# Autodesk Inventor assembly: Framework_Link_COG
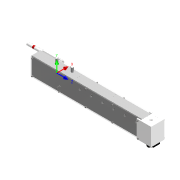
[picture p0: Inventor's stored thumbnail of the model, 180x180]
Saved by Autodesk Inventor 2022 (Build 260153000, 153)
## iProperties
Created: 2022-10-18
Part Number: Framework_Link_COG
Document SubType Name: Assembly
Designer: alexw
Mass: 1238.25 g
Surface Area: 4599.21 cm^2
Volume: 1168.94 cm^3
Density: 1.05929 g/cm^3
Author: alexw
## Documents named in this file (17)
- C:\Users\alexw\Documents\Inventor\Projects\03_CurrentProjects\MasterThesis\PSM_V1_Rillenkugellager\COG\Framework_Link_COG.iam
- C:\Users\alexw\Documents\Inventor\Projects\03_CurrentProjects\MasterThesis\PSM_V1_Rillenkugellager\Ueberarbeiteter DaVincikopf\Fuehrungsschiene.ipt
- C:\Users\alexw\Documents\Inventor\Projects\03_CurrentProjects\MasterThesis\PSM_V1_Rillenkugellager\Back plate profile.ipt
- C:\Users\alexw\Documents\Inventor\Projects\03_CurrentProjects\MasterThesis\PSM_V1_Rillenkugellager\Slot profile.ipt
- C:\Users\alexw\Documents\Inventor\Projects\03_CurrentProjects\MasterThesis\PSM_V1_Rillenkugellager\Guide.ipt
- C:\Users\alexw\Documents\Inventor\Projects\03_CurrentProjects\MasterThesis\PSM_V1_Rillenkugellager\Ueberarbeiteter DaVincikopf\Zahnradbahn.ipt
- C:\Users\alexw\Documents\Inventor\Projects\03_CurrentProjects\MasterThesis\PSM_V1_Rillenkugellager\ContentCenter\de-DE\ISO 4762(2)\ISO 4762 - M3 x 10ISO.ipt
- C:\Users\alexw\Documents\Inventor\Projects\03_CurrentProjects\MasterThesis\PSM_V1_Rillenkugellager\ContentCenter\de-DE\ISO 4762(2)\ISO 4762 - M3 x 12ISO.ipt
- C:\Users\alexw\Documents\Inventor\Projects\03_CurrentProjects\MasterThesis\PSM_V1_Rillenkugellager\ContentCenter\de-DE\ISO 10642(1)\ISO 10642 - M3 x  8.ipt
- C:\Users\alexw\Documents\Inventor\Projects\03_CurrentProjects\MasterThesis\PSM_V1_Rillenkugellager\ContentCenter\de-DE\ISO 4762(2)\ISO 4762 - M3 x 16ISO.ipt
- C:\Users\alexw\Documents\Inventor\Projects\03_CurrentProjects\MasterThesis\PSM_V1_Rillenkugellager\Riemenspanner_Bottompart_Assembly.iam
- C:\Users\alexw\Documents\Inventor\Projects\03_CurrentProjects\MasterThesis\PSM_V1_Rillenkugellager\Sensor_Box_Assembly.ipt.iam
- C:\Users\alexw\Documents\Inventor\Projects\03_CurrentProjects\MasterThesis\PSM_V1_Rillenkugellager\ContentCenter\de-DE\ISO 4762(2)\ISO 4762 - M3 x 20ISO.ipt
- C:\Users\alexw\Documents\Inventor\Projects\03_CurrentProjects\MasterThesis\PSM_V1_Rillenkugellager\Riemen_T5.ipt
- C:\Users\alexw\Documents\Inventor\Projects\03_CurrentProjects\MasterThesis\PSM_V1_Rillenkugellager\ContentCenter\de-DE\ISO 4762(2)\ISO 4762 - M5 x 25ISO.ipt
- C:\Users\alexw\Documents\Inventor\Projects\03_CurrentProjects\MasterThesis\PSM_V1_Rillenkugellager\10_79_0000_0010_003.ipt
- Sensor_Box_Assembly.ipt
## Components (43 placed, 15 different names)
1. Fuehrungsschiene:1 — Passend:73, Passend:74, Passend:75, Passend:76, Passend:77, Passend:78, Passend:79, Passend:80, Fluchtend:3
2. Back plate profile:1 — Winkel:1
3. Slot profile:1
4. Guide:1
5. Zahnradbahn:1
6. ISO 4762 M3 x 10:1
7. ISO 4762 M3 x 10:2
8. ISO 4762 M3 x 10:3
9. ISO 4762 M3 x 10:4
10. ISO 4762 M3 x 10:5
11. ISO 4762 M3 x 10:6
12. ISO 4762 M3 x 10:7
13. ISO 4762 M3 x 10:8
14. ISO 4762 M3 x 12:1
15. ISO 4762 M3 x 12:2
16. ISO 4762 M3 x 12:3
17. ISO 4762 M3 x 12:4
18. ISO 4762 M3 x 12:5
19. ISO 4762 M3 x 12:6
20. ISO 10642 M3x8:1
21. ISO 10642 M3x8:2
22. ISO 10642 M3x8:3
23. ISO 10642 M3x8:4
24. ISO 10642 M3x8:5
25. ISO 10642 M3x8:6
26. ISO 4762 M3 x 16:1
27. ISO 4762 M3 x 16:2
28. ISO 4762 M3 x 16:3
29. ISO 4762 M3 x 16:4
30. Riemenspanner_Bottompart_Assembly:1 [sub-assembly] — Passend:83
31. Sensor_Box_Assembly.ipt:1 [sub-assembly] — Passend:84
32. ISO 4762 M3 x 20:1
33. ISO 4762 M3 x 20:2
34. ISO 4762 M3 x 20:3
35. ISO 4762 M3 x 20:4
36. ISO 4762 M3 x 16:5
37. ISO 4762 M3 x 16:6
38. Riemen_T5:1 — Passend:83, Passend:84
39. ISO 4762 M5 x 25:1
40. 10_79_0000_0010_003:1 — Passend:73, Passend:79
41. 10_79_0000_0010_003:2 — Passend:74, Passend:80, Passend:81, Passend:82
42. 10_79_0000_0010_003:3 — Passend:75, Passend:77
43. 10_79_0000_0010_003:4 — Passend:76, Passend:78
## Relationships (88: Mate 84, Flush 3, Angle 1)
- [Mate]: Fuehrungsschiene:1 ↔ Slot profile:1
- [Mate]: Slot profile:1 ↔ Guide:1
- [Mate]: Fuehrungsschiene:1 ↔ ISO 4762 M3 x 10:1
- [Mate]: Back plate profile:1 ↔ ISO 4762 M3 x 10:1
- [Mate]: Fuehrungsschiene:1 ↔ ISO 4762 M3 x 10:2
- [Mate]: Back plate profile:1 ↔ ISO 4762 M3 x 10:2
- [Mate]: Fuehrungsschiene:1 ↔ ISO 4762 M3 x 10:3
- [Mate]: Back plate profile:1 ↔ ISO 4762 M3 x 10:3
- [Mate]: Fuehrungsschiene:1 ↔ ISO 4762 M3 x 10:4
- [Mate]: Back plate profile:1 ↔ ISO 4762 M3 x 10:4
- [Mate]: Fuehrungsschiene:1 ↔ ISO 4762 M3 x 10:5
- [Mate]: Back plate profile:1 ↔ ISO 4762 M3 x 10:5
- [Mate]: Fuehrungsschiene:1 ↔ ISO 4762 M3 x 10:6
- [Mate]: Back plate profile:1 ↔ ISO 4762 M3 x 10:6
- [Mate]: Fuehrungsschiene:1 ↔ ISO 4762 M3 x 10:7
- [Mate]: Back plate profile:1 ↔ ISO 4762 M3 x 10:7
- [Mate]: Fuehrungsschiene:1 ↔ ISO 4762 M3 x 10:8
- [Mate]: Back plate profile:1 ↔ ISO 4762 M3 x 10:8
- [Mate]: Fuehrungsschiene:1 ↔ ISO 4762 M3 x 12:1
- [Mate]: Slot profile:1 ↔ ISO 4762 M3 x 12:1
- [Mate]: Fuehrungsschiene:1 ↔ ISO 4762 M3 x 12:2
- [Mate]: Slot profile:1 ↔ ISO 4762 M3 x 12:2
- [Mate]: Fuehrungsschiene:1 ↔ ISO 4762 M3 x 12:3
- [Mate]: Slot profile:1 ↔ ISO 4762 M3 x 12:3
- [Mate]: Fuehrungsschiene:1 ↔ ISO 4762 M3 x 12:4
- [Mate]: Slot profile:1 ↔ ISO 4762 M3 x 12:4
- [Mate]: Fuehrungsschiene:1 ↔ ISO 4762 M3 x 12:5
- [Mate]: Slot profile:1 ↔ ISO 4762 M3 x 12:5
- [Mate]: Fuehrungsschiene:1 ↔ ISO 4762 M3 x 12:6
- [Mate]: Slot profile:1 ↔ ISO 4762 M3 x 12:6
- [Mate]: Fuehrungsschiene:1 ↔ Back plate profile:1
- [Mate]: Back plate profile:1 ↔ ISO 4762 M3 x 10:7
- [Mate]: Fuehrungsschiene:1 ↔ Slot profile:1
- [Mate]: Fuehrungsschiene:1 ↔ ISO 10642 M3x8:1
- [Mate]: Fuehrungsschiene:1 ↔ ISO 10642 M3x8:2
- [Mate]: Fuehrungsschiene:1 ↔ ISO 10642 M3x8:3
- [Mate]: Fuehrungsschiene:1 ↔ ISO 10642 M3x8:4
- [Mate]: Fuehrungsschiene:1 ↔ ISO 10642 M3x8:5
- [Mate]: Fuehrungsschiene:1 ↔ ISO 10642 M3x8:6
- [Mate]: Slot profile:1 ↔ Guide:1
- [Mate]: Slot profile:1 ↔ Guide:1
- [Mate]: Fuehrungsschiene:1 ↔ Zahnradbahn:1
- [Flush]: Fuehrungsschiene:1 ↔ Zahnradbahn:1
- [Mate]: Fuehrungsschiene:1 ↔ Zahnradbahn:1
- [Mate]: Fuehrungsschiene:1 ↔ Zahnradbahn:1
- [Mate]: Guide:1 ↔ ISO 4762 M3 x 16:1
- [Mate]: Guide:1 ↔ ISO 4762 M3 x 16:1
- [Mate]: Guide:1 ↔ ISO 4762 M3 x 16:2
- [Mate]: Guide:1 ↔ ISO 4762 M3 x 16:2
- [Mate]: Guide:1 ↔ ISO 4762 M3 x 16:3
- [Mate]: Guide:1 ↔ ISO 4762 M3 x 16:3
- [Mate]: Guide:1 ↔ ISO 4762 M3 x 16:4
- [Mate]: Guide:1 ↔ ISO 4762 M3 x 16:4
- [Mate]: Fuehrungsschiene:1 ↔ Riemenspanner_Bottompart_Assembly:1
- [Mate]: Fuehrungsschiene:1 ↔ Riemenspanner_Bottompart_Assembly:1
- [Mate]: Back plate profile:1 ↔ Sensor_Box_Assembly.ipt:1
- [Mate]: Fuehrungsschiene:1 ↔ Sensor_Box_Assembly.ipt:1
- [Mate]: Slot profile:1 ↔ Sensor_Box_Assembly.ipt:1
- [Mate]: Fuehrungsschiene:1 ↔ ISO 4762 M3 x 20:1
- [Mate]: Sensor_Box_Assembly.ipt:1 ↔ ISO 4762 M3 x 20:1
- [Mate]: Sensor_Box_Assembly.ipt:1 ↔ ISO 4762 M3 x 20:2
- [Mate]: Sensor_Box_Assembly.ipt:1 ↔ ISO 4762 M3 x 20:2
- [Mate]: Sensor_Box_Assembly.ipt:1 ↔ ISO 4762 M3 x 20:3
- [Mate]: Sensor_Box_Assembly.ipt:1 ↔ ISO 4762 M3 x 20:3
- [Mate]: Sensor_Box_Assembly.ipt:1 ↔ ISO 4762 M3 x 20:4
- [Mate]: Sensor_Box_Assembly.ipt:1 ↔ ISO 4762 M3 x 20:4
- [Mate]: Sensor_Box_Assembly.ipt:1 ↔ ISO 4762 M3 x 16:5
- [Mate]: Sensor_Box_Assembly.ipt:1 ↔ ISO 4762 M3 x 16:5
- [Mate]: Sensor_Box_Assembly.ipt:1 ↔ ISO 4762 M3 x 16:6
- [Mate]: Sensor_Box_Assembly.ipt:1 ↔ ISO 4762 M3 x 16:6
- [Mate] (370 mm): Riemenspanner_Bottompart_Assembly:1 ↔ Sensor_Box_Assembly.ipt:1
- [Mate]: Fuehrungsschiene:1 ↔ ISO 4762 M5 x 25:1
- [Mate]: Riemenspanner_Bottompart_Assembly:1 ↔ ISO 4762 M5 x 25:1
- [Flush]: Sensor_Box_Assembly.ipt:1 ↔ Riemen_T5:1
- Passend:73 [Mate]: Fuehrungsschiene:1 ↔ 10_79_0000_0010_003:1
- Passend:74 [Mate]: Fuehrungsschiene:1 ↔ 10_79_0000_0010_003:2
- Passend:75 [Mate]: Fuehrungsschiene:1 ↔ 10_79_0000_0010_003:3
- Passend:76 [Mate]: Fuehrungsschiene:1 ↔ 10_79_0000_0010_003:4
- Passend:77 [Mate]: Fuehrungsschiene:1 ↔ 10_79_0000_0010_003:3
- Passend:78 [Mate]: Fuehrungsschiene:1 ↔ 10_79_0000_0010_003:4
- Passend:79 [Mate]: Fuehrungsschiene:1 ↔ 10_79_0000_0010_003:1
- Passend:80 [Mate]: Fuehrungsschiene:1 ↔ 10_79_0000_0010_003:2
- Passend:81 [Mate]: 10_79_0000_0010_003:2
- Passend:82 [Mate]: 10_79_0000_0010_003:2
- Winkel:1 [Angle] (0 deg): Back plate profile:1
- Passend:83 [Mate]: Riemenspanner_Bottompart_Assembly:1 ↔ Riemen_T5:1
- Passend:84 [Mate]: Sensor_Box_Assembly.ipt:1 ↔ Riemen_T5:1
- Fluchtend:3 [Flush]: Fuehrungsschiene:1
## Named parameters: d85_d117 = 0 mm, d86_d118 = 0 mm, d87_d119 = 0 mm, d88_d120 = 0 mm, d89_d121 = 0 mm, d90_d122 = 0 mm, d91_d123 = 0 mm, d92_d124 = 0 mm, d93_d125 = 0 mm, d94_d126 = 0 mm, d95_d127 = 0 mm, d96_d128 = 0 mm, d97_d129 = 0 mm, d98_d130 = 0 mm, d99_d131 = 0 mm, d100_d132 = 0 mm, d101_d133 = 0 mm, d102_d134 = 0 mm, d103_d135 = 0 mm
